# Autodesk Inventor assembly: 092_CPY
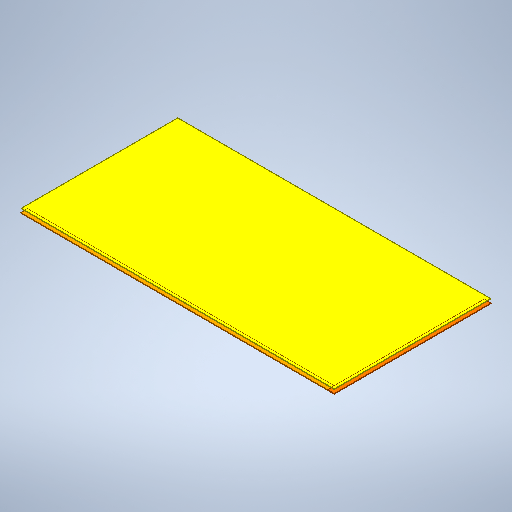
[picture p0: Inventor's stored thumbnail of the model, 512x512]
Saved by Autodesk Inventor 2026.2 (Build 302298000, 298)
## iProperties
Created: 2026-05-19
Part Number: 092_CPY
Document SubType Name: Assembly
Designer: user
Author: user
## Documents named in this file (4)
- C:\Users\admin\Documents\Inventor\GBK-Gubkinskiy\092_CPY.iam
- C:\Users\admin\Documents\Inventor\GBK-Gubkinskiy\0921_CPY.ipt
- C:\Users\admin\Documents\Inventor\GBK-Gubkinskiy\0922_CPY.ipt
- C:\Users\admin\Documents\Inventor\GBK-Gubkinskiy\0923_CPY.ipt
## Components (3 placed, 3 different names)
1. 0921_CPY:1 — Flush:1, Mate:1, Flush:2
2. 0922_CPY:1 — Flush:1, Mate:1, Rigid:1
3. 0923_CPY:1 — Flush:2, Rigid:1
## Relationships (4: Flush 2, Mate 1, WeldJoint 1)
- Flush:1 (34 mm): 0921_CPY:1 ↔ 0922_CPY:1
- Mate:1: 0921_CPY:1 ↔ 0922_CPY:1
- Flush:2 (34 mm): 0921_CPY:1 ↔ 0923_CPY:1
- Rigid:1 [WeldJoint]: 0922_CPY:1 ↔ 0923_CPY:1
